# Autodesk Inventor assembly: RGBLed bent
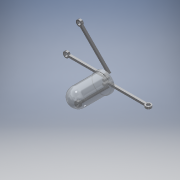
[picture p0: Inventor's stored thumbnail of the model, 180x180]
Saved by Autodesk Inventor 2019.3 (Build 233278000, 278)
## iProperties
Created: 2019-01-07
Part Number: RGBLed bent
Material: Generisch
Document SubType Name: Assembly
Designer: Jonas
Author: Jonas
## Documents named in this file (4)
- C:\Users\Jonas\Desktop\RGBCube\RGBCubev2\CAD\Led\RGBLed bent.iam
- C:\Users\Jonas\Desktop\RGBCube\RGBCubev2\CAD\Led\Head.ipt
- C:\Users\Jonas\Desktop\RGBCube\RGBCubev2\CAD\Led\LegCathode.ipt
- C:\Users\Jonas\Desktop\RGBCube\RGBCubev2\CAD\Led\LegAnode.ipt
## Components (5 placed, 3 different names)
1. Head:1 — Passend:1, Tangential:1, Passend:3, Passend:4, Passend:5, Tangential:2, Passend:14
2. LegCathode:1 — Passend:1, Passend:2, Passend:6, Passend:7, Passend:10, Winkel:4
3. LegAnode:1 — Passend:3, Passend:9, Passend:13
4. LegAnode:2 — Passend:4, Fluchtend:1, Passend:6, Passend:8, Winkel:3
5. LegAnode:3 — Passend:5, Passend:11, Passend:12
## Relationships (21: Mate 14, Angle 4, Tangent 2, Flush 1)
- Passend:1 [Mate] (-0.5 mm): Head:1 ↔ LegCathode:1
- Winkel:1 [Angle] (0 deg)
- Tangential:1 (-2.55 mm): Head:1
- Passend:2 [Mate] (-0.3 mm): LegCathode:1
- Passend:3 [Mate] (-0.5 mm): Head:1 ↔ LegAnode:1
- Passend:4 [Mate] (-0.5 mm): Head:1 ↔ LegAnode:2
- Passend:5 [Mate] (-0.5 mm): Head:1 ↔ LegAnode:3
- Fluchtend:1 [Flush] (-0.3 mm): LegAnode:2
- Passend:6 [Mate] (0.5 mm): LegCathode:1 ↔ LegAnode:2
- Winkel:2 [Angle] (0 deg)
- Tangential:2: Head:1
- Passend:7 [Mate] (-3.6 mm): LegCathode:1
- Passend:8 [Mate]: LegAnode:2
- Winkel:3 [Angle] (45 deg): LegAnode:2
- Passend:9 [Mate] (0.5 mm): LegAnode:1
- Passend:10 [Mate]: LegCathode:1
- Winkel:4 [Angle] (-45 deg): LegCathode:1
- Passend:11 [Mate] (0.5 mm): LegAnode:3
- Passend:12 [Mate] (-0.2 mm): LegAnode:3
- Passend:13 [Mate] (0.3 mm): LegAnode:1
- Passend:14 [Mate]: Head:1
